# Autodesk Inventor assembly: Robot_Arm
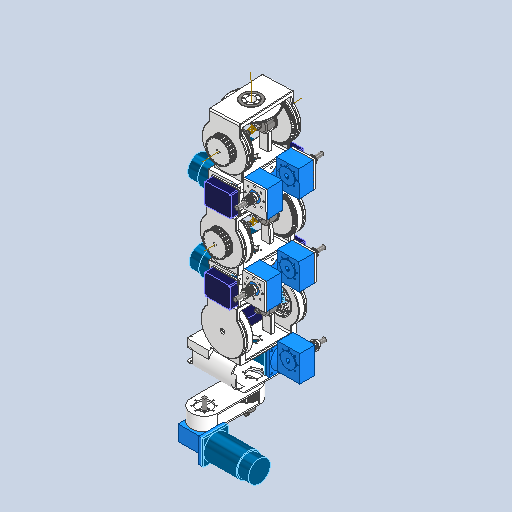
[picture p0: Inventor's stored thumbnail of the model, 512x512]
Saved by Autodesk Inventor 2025.3 (Build 293356030, 356C)
## iProperties
Created: 2025-09-07
Part Number: Robot_Arm
Document SubType Name: Assembly
Designer: MSI
Mass: 32952.7 g
Surface Area: 29125.4 cm^2
Volume: 17434.5 cm^3
Density: 1.89009 g/cm^3
Author: MSI
## Documents named in this file (5)
- C:\Users\MSI\Desktop\Project\3. 로봇팔\Robot Arm Model\Robot_Arm_6_v1\Robot_Arm.iam
- C:\Users\MSI\Desktop\Project\3. 로봇팔\Robot Arm Model\Robot_Arm_6_v1\joint1.iam
- C:\Users\MSI\Desktop\Project\3. 로봇팔\Robot Arm Model\Robot_Arm_6_v1\joint2.iam
- C:\Users\MSI\Desktop\Project\3. 로봇팔\Robot Arm Model\Robot_Arm_6_v1\joint3.iam
- C:\Users\MSI\Desktop\Project\3. 로봇팔\Robot Arm Model\Robot_Arm_6_v1\joint4.iam
## Components (4 placed, 4 different names)
1. joint1:1 [sub-assembly] — 회전:4
2. joint2:1 [sub-assembly] — 회전:4, 강체:4
3. joint3:1 [sub-assembly] — 강체:4, 강체:3
4. joint4:1 [sub-assembly] — 강체:3
## Relationships (3: WeldJoint 2, RevoluteJoint 1)
- 회전:4 [RevoluteJoint]: joint1:1 ↔ joint2:1
- 강체:4 [WeldJoint]: joint2:1 ↔ joint3:1
- 강체:3 [WeldJoint]: joint3:1 ↔ joint4:1
